# Autodesk Inventor assembly: HERRAMIENTA
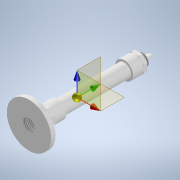
[picture p0: Inventor's stored thumbnail of the model, 180x180]
Saved by Autodesk Inventor 2022 (Build 260153000, 153)
## iProperties
Created: 2022-09-01
Part Number: HERRAMIENTA
Document SubType Name: Assembly
Designer: Usuario
Mass: 160 g
Surface Area: 461.668 cm^2
Volume: 76.1228 cm^3
Author: Usuario
## Documents named in this file (6)
- C:\Users\Usuario\Documents\Cosas de Sebastian\Robotica\LAB\LAB1\HERRAMIENTA\HERRAMIENTA.iam
- C:\Users\Usuario\Documents\Cosas de Sebastian\Robotica\LAB\LAB1\HERRAMIENTA\ACOPLE.ipt
- C:\Users\Usuario\Documents\Cosas de Sebastian\Robotica\LAB\LAB1\HERRAMIENTA\FLANCHE.ipt
- C:\Users\Usuario\Documents\Cosas de Sebastian\Robotica\LAB\LAB1\HERRAMIENTA\TUBO.ipt
- C:\Users\Usuario\Documents\Cosas de Sebastian\Robotica\LAB\LAB1\HERRAMIENTA\ACOPLE2.ipt
- C:\Users\Usuario\Documents\Cosas de Sebastian\Robotica\LAB\LAB1\HERRAMIENTA\MARCADOR.ipt
## Components (5 placed, 5 different names)
1. ACOPLE:1 — Coincidencia:1, Insertar:1, Coincidencia:3
2. FLANCHE:1 — Coincidencia:1, Coincidencia:2, Nivelación:1, Coincidencia:3
3. TUBO:1 — Insertar:1, Rígido:1
4. ACOPLE2:1 — Insertar:2, Rígido:1
5. MARCADOR:1 — Insertar:2
## Relationships (7: Mate 3, Insert 2, WeldJoint 1, Flush 1)
- Coincidencia:1 [Mate]: ACOPLE:1 ↔ FLANCHE:1
- Insertar:1: ACOPLE:1 ↔ TUBO:1
- Insertar:2 (-4.42 mm): ACOPLE2:1 ↔ MARCADOR:1
- Rígido:1 [WeldJoint] (-18.44 mm): TUBO:1 ↔ ACOPLE2:1
- Coincidencia:2 [Mate]: FLANCHE:1
- Nivelación:1 [Flush]: FLANCHE:1
- Coincidencia:3 [Mate]: ACOPLE:1 ↔ FLANCHE:1
